# Autodesk Inventor assembly: Assembly1
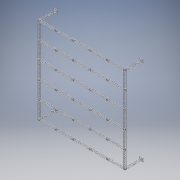
[picture p0: Inventor's stored thumbnail of the model, 180x180]
Saved by Autodesk Inventor 2019 (Build 230136000, 136)
## iProperties
Created: 2017-07-14
Part Number: Assembly1
Document SubType Name: Assembly
Designer: close
Sending System: Autodesk Inventor 2017
Preprocessor: ST-DEVELOPER v16.5
Title: C:\Users\Kledson\Downloads\PROJETO K\Estrutura metalica - Metal structure\BOXTruss\T30\Assembly1.stp
Author: Kledson
## Documents named in this file (5)
- C:\Users\close\Desktop\BARC-ROAR\barc_hardware\Dependencies\truss rails\50ft.iam
- C:\Users\close\Desktop\BARC-ROAR\barc_hardware\Dependencies\truss rails\Base 700x700.iam
- C:\Users\close\Desktop\BARC-ROAR\barc_hardware\Dependencies\truss rails\Coluna3000.ipt.iam
- C:\Users\close\Desktop\BARC-ROAR\barc_hardware\Dependencies\truss rails\Box 300x300.iam
- Coluna3000.ipt
## Components (84 placed, 3 different names)
1. Coluna3000.ipt:3 [sub-assembly]
2. Coluna3000.ipt:9 [sub-assembly]
3. Coluna3000.ipt:10 [sub-assembly]
4. Coluna3000.ipt:11 [sub-assembly]
5. Coluna3000.ipt:12 [sub-assembly]
6. Coluna3000.ipt:13 [sub-assembly]
7. Coluna3000.ipt:14 [sub-assembly]
8. Coluna3000.ipt:15 [sub-assembly]
9. Coluna3000.ipt:16 [sub-assembly]
10. Coluna3000.ipt:17 [sub-assembly]
11. Coluna3000.ipt:18 [sub-assembly]
12. Coluna3000.ipt:19 [sub-assembly]
13. Coluna3000.ipt:20 [sub-assembly]
14. Coluna3000.ipt:21 [sub-assembly]
15. Coluna3000.ipt:22 [sub-assembly]
16. Coluna3000.ipt:23 [sub-assembly]
17. Coluna3000.ipt:24 [sub-assembly]
18. Coluna3000.ipt:25 [sub-assembly]
19. Coluna3000.ipt:26 [sub-assembly]
20. Coluna3000.ipt:27 [sub-assembly]
21. Coluna3000.ipt:28 [sub-assembly]
22. Coluna3000.ipt:29 [sub-assembly]
23. Coluna3000.ipt:30 [sub-assembly]
24. Coluna3000.ipt:31 [sub-assembly]
25. Coluna3000.ipt:32 [sub-assembly]
26. Coluna3000.ipt:62 [sub-assembly]
27. Coluna3000.ipt:63 [sub-assembly]
28. Coluna3000.ipt:64 [sub-assembly]
29. Coluna3000.ipt:65 [sub-assembly]
30. Coluna3000.ipt:66 [sub-assembly]
31. Coluna3000.ipt:8 [sub-assembly]
32. Coluna3000.ipt:33 [sub-assembly]
33. Coluna3000.ipt:34 [sub-assembly]
34. Coluna3000.ipt:35 [sub-assembly]
35. Coluna3000.ipt:36 [sub-assembly]
36. Coluna3000.ipt:37 [sub-assembly]
37. Coluna3000.ipt:38 [sub-assembly]
38. Coluna3000.ipt:39 [sub-assembly]
39. Coluna3000.ipt:40 [sub-assembly]
40. Coluna3000.ipt:41 [sub-assembly]
41. Box 300x300:3 [sub-assembly]
42. Box 300x300:4 [sub-assembly]
43. Box 300x300:5 [sub-assembly]
44. Box 300x300:6 [sub-assembly]
45. Box 300x300:7 [sub-assembly]
46. Box 300x300:8 [sub-assembly]
47. Box 300x300:9 [sub-assembly]
48. Box 300x300:10 [sub-assembly]
49. Box 300x300:11 [sub-assembly]
50. Box 300x300:12 [sub-assembly]
51. Box 300x300:13 [sub-assembly]
52. Box 300x300:14 [sub-assembly]
53. Box 300x300:15 [sub-assembly]
54. Box 300x300:16 [sub-assembly]
55. Box 300x300:17 [sub-assembly]
56. Box 300x300:18 [sub-assembly]
57. Box 300x300:19 [sub-assembly]
58. Box 300x300:20 [sub-assembly]
59. Box 300x300:21 [sub-assembly]
60. Box 300x300:22 [sub-assembly]
61. Box 300x300:23 [sub-assembly]
62. Box 300x300:24 [sub-assembly]
63. Box 300x300:25 [sub-assembly]
64. Box 300x300:26 [sub-assembly]
65. Box 300x300:27 [sub-assembly]
66. Box 300x300:28 [sub-assembly]
67. Box 300x300:29 [sub-assembly]
68. Box 300x300:30 [sub-assembly]
69. Box 300x300:31 [sub-assembly]
70. Box 300x300:32 [sub-assembly]
71. Box 300x300:33 [sub-assembly]
72. Box 300x300:34 [sub-assembly]
73. Box 300x300:35 [sub-assembly]
74. Box 300x300:36 [sub-assembly]
75. Box 300x300:37 [sub-assembly]
76. Box 300x300:38 [sub-assembly]
77. Coluna3000.ipt:4 [sub-assembly]
78. Base 700x700:2 [sub-assembly]
79. Coluna3000.ipt:67 [sub-assembly]
80. Base 700x700:3 [sub-assembly]
81. Coluna3000.ipt:68 [sub-assembly]
82. Base 700x700:4 [sub-assembly]
83. Coluna3000.ipt:69 [sub-assembly]
84. Base 700x700:5 [sub-assembly]
## Component patterns: (30 elements, first: Coluna3000.ipt:3), (10 elements, first: Coluna3000.ipt:8), (36 elements, first: Box 300x300:3), (4 elements, first: Coluna3000.ipt:4 + Base 700x700:2)
